# Autodesk Inventor assembly: Assembly1
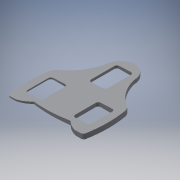
[picture p0: Inventor's stored thumbnail of the model, 180x180]
Saved by Autodesk Inventor 2019 (Build 230136000, 136)
## iProperties
Created: 2019-06-08
Part Number: Assembly1
Document SubType Name: Assembly
Designer: assman
Author: assman
## Documents named in this file (4)
- D:\Inventor\Projects\Calas Carretera\Assembly1.iam
- D:\Inventor\Projects\Calas Carretera\shim_3_mm.ipt
- D:\Inventor\Projects\Calas Carretera\cutaway_1mm.ipt
- D:\Inventor\Projects\Calas Carretera\shim_3mm_cut.ipt
## Components (3 placed, 3 different names)
1. shim_3mm_cut:1
2. shim_3_mm:1 — Rigid:1
3. cutaway_1mm:1 — Rigid:1
## Relationships (1: WeldJoint 1)
- Rigid:1 [WeldJoint] (-30 mm): shim_3_mm:1 ↔ cutaway_1mm:1
